# Autodesk Inventor assembly: MODI
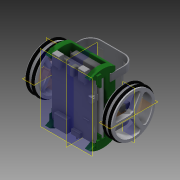
[picture p0: Inventor's stored thumbnail of the model, 180x180]
Saved by Autodesk Inventor 2013 (Build 170138000, 138)
## iProperties
Created: 2013-04-30
Part Number: MODI
Document SubType Name: Assembly
Designer: otrab
Author: otrab
## Documents named in this file (11)
- C:\Users\otrab\Documents\GitHub\modi\Hardware\inventor 2013\MODI.iam
- C:\Users\otrab\Documents\GitHub\modi\Hardware\inventor 2013\Chasis.ipt
- C:\Users\otrab\Documents\GitHub\modi\Hardware\inventor 2013\bateria.ipt
- C:\Users\otrab\Documents\GitHub\modi\Hardware\inventor 2013\fio.ipt
- C:\Users\otrab\Documents\GitHub\modi\Hardware\inventor 2013\lipoRiderPro.ipt
- C:\Users\otrab\Documents\GitHub\modi\Hardware\inventor 2013\Rueda.ipt
- C:\Users\otrab\Documents\GitHub\modi\Hardware\inventor 2013\tapa.ipt
- C:\Users\otrab\Documents\GitHub\modi\Hardware\inventor 2013\Adaptador TB6612FNG.ipt
- C:\Users\otrab\Documents\GitHub\modi\Hardware\inventor 2013\motor pololu.ipt
- C:\Users\otrab\Documents\GitHub\modi\Hardware\inventor 2013\orings.ipt
- C:\Users\otrab\Documents\GitHub\modi\Hardware\inventor 2013\SoporteFio.ipt
## Components (15 placed, 10 different names)
1. Chasis:1 — Mate:3, Mate:4, Insert:1, Insert:2
2. bateria:1
3. fio:1 — Mate:3, Mate:4
4. lipoRiderPro:1
5. Rueda:1 — Mate:5
6. Rueda:2 — Mate:6
7. tapa:1
8. Adaptador TB6612FNG:1
9. motor pololu:1 — Insert:1, Mate:6
10. motor pololu:2 — Insert:2, Mate:5
11. orings:1
12. SoporteFio:1
13. orings:2
14. orings:3
15. orings:4
## Relationships (6: Mate 4, Insert 2)
- Mate:3: Chasis:1 ↔ fio:1
- Mate:4: Chasis:1 ↔ fio:1
- Insert:1: Chasis:1 ↔ motor pololu:1
- Insert:2: Chasis:1 ↔ motor pololu:2
- Mate:5: Rueda:1 ↔ motor pololu:2
- Mate:6: Rueda:2 ↔ motor pololu:1
